# Autodesk Inventor assembly: ViseAAssembly
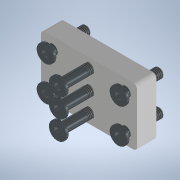
[picture p0: Inventor's stored thumbnail of the model, 180x180]
Saved by Autodesk Inventor 2022 (Build 260153000, 153)
## iProperties
Created: 2021-11-10
Part Number: ViseAAssembly
Document SubType Name: Assembly
Designer: JK
Author: JK
## Documents named in this file (5)
- C:\Users\JK\Documents\Inventor\UTM\ViseAAssembly.iam
- C:\Users\JK\Documents\Inventor\UTM\ViseA.ipt
- C:\Users\JK\Documents\Inventor\UTM\M5Nut.ipt
- C:\Users\JK\Documents\Inventor\UTM\PernoM5x25Plano.ipt
- C:\Users\JK\Documents\Inventor\UTM\M5x20BoltFlatHead.ipt
## Components (15 placed, 4 different names)
1. ViseA:1 — Coincidencia:3, Coincidencia:4, Coincidencia:5, Ángulo:2, Coincidencia:6, Coincidencia:7
2. PernoM5x25Plano:1 — Coincidencia:3, Coincidencia:4
3. M5Nut:1
4. PernoM5x25Plano:2
5. M5Nut:2
6. PernoM5x25Plano:3
7. M5Nut:3
8. M5Nut:4 — Coincidencia:5, Ángulo:2, Coincidencia:6
9. M5Nut:5
10. M5Nut:6
11. M5Nut:7
12. M5x20BoltFlatHead:1 — Coincidencia:7
13. M5x20BoltFlatHead:2
14. M5x20BoltFlatHead:3
15. M5x20BoltFlatHead:4
## Component patterns: (3 elements, first: PernoM5x25Plano:1 + M5Nut:1), (4 elements, first: M5Nut:4), (4 elements, first: M5x20BoltFlatHead:1)
## Relationships (9: Mate 7, Angle 2)
- [Mate]: ViseA:1 ↔ M5Nut:1
- [Angle] (0 deg): ViseA:1 ↔ M5Nut:1
- [Mate]: ViseA:1 ↔ M5Nut:1
- Coincidencia:3 [Mate]: ViseA:1 ↔ PernoM5x25Plano:1
- Coincidencia:4 [Mate] (15 mm): ViseA:1 ↔ PernoM5x25Plano:1
- Coincidencia:5 [Mate]: ViseA:1 ↔ M5Nut:4
- Ángulo:2 [Angle] (0 deg): ViseA:1 ↔ M5Nut:4
- Coincidencia:6 [Mate]: ViseA:1 ↔ M5Nut:4
- Coincidencia:7 [Mate]: ViseA:1 ↔ M5x20BoltFlatHead:1
